# Autodesk Inventor assembly: parachute_structure_asm
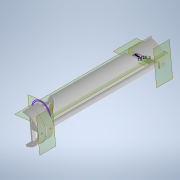
[picture p0: Inventor's stored thumbnail of the model, 180x180]
Saved by Autodesk Inventor 2020 (Build 240168000, 168)
## iProperties
Created: 2022-03-10
Part Number: parachute_structure_asm
Document SubType Name: Assembly
Designer: sp
Author: sp
## Documents named in this file (5)
- C:\Users\sp\Documents\Rocket\rocket\CAD\parachute_structure_asm.iam
- C:\Users\sp\Documents\Rocket\rocket\CAD\stange.ipt
- C:\Users\sp\Documents\Rocket\rocket\CAD\Verbindungsring_2_2.ipt
- C:\Users\sp\Documents\Rocket\rocket\CAD\Verbindungsring_2_3.ipt
- C:\Users\sp\Documents\Rocket\rocket\CAD\Parachute_In.ipt
## Components (5 placed, 4 different names)
1. stange:1 — Einfügen:1, Einfügen:3
2. stange:2 — Einfügen:2, Einfügen:4, Tangential:1
3. Verbindungsring_2_2:1 — Einfügen:1, Einfügen:2
4. Parachute_In:1 — Tangential:1
5. Verbindungsring_2_3:1 — Einfügen:3, Einfügen:4
## Relationships (5: Insert 4, Tangent 1)
- Einfügen:1 [Insert]: stange:1 ↔ Verbindungsring_2_2:1
- Einfügen:2 [Insert]: stange:2 ↔ Verbindungsring_2_2:1
- Einfügen:3 [Insert]: stange:1 ↔ Verbindungsring_2_3:1
- Einfügen:4 [Insert]: stange:2 ↔ Verbindungsring_2_3:1
- Tangential:1: stange:2 ↔ Parachute_In:1
